# Autodesk Inventor assembly: IntakeExtensionBar
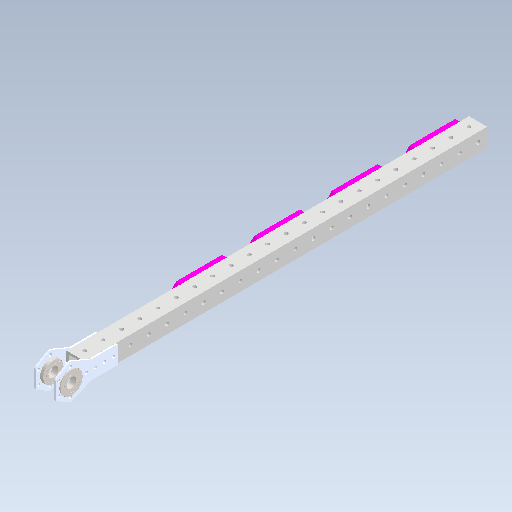
[picture p0: Inventor's stored thumbnail of the model, 512x512]
Saved by Autodesk Inventor 2020 (Build 240168000, 168)
## iProperties
Created: 2020-01-19
Part Number: IntakeExtensionBar
Document SubType Name: Assembly
Designer: srini
Author: srini
## Documents named in this file (5)
- C:\Users\srini\Documents\FRC\2020\IntakeShooter\IntakeExtensionBar.iam
- C:\Users\srini\Documents\FRC\2020\IntakeShooter\1x1x18.ipt
- C:\Users\srini\Documents\FRC\2020\IntakeShooter\VersaFrame_End_Bearing_Gusset_217-3554.ipt
- C:\Users\srini\Documents\FRC\2020\IntakeShooter\13_75mm_1_2_ThunderHex_ID_x_1_125_OD_x_0_313_WD_Flanged_Bearing_217-4006.ipt
- C:\Users\srini\Documents\FRC\2020\IntakeShooter\ShaftRest.ipt
## Components (9 placed, 4 different names)
1. 1x1x18:1 — Insert:7, Insert:8, Insert:9, Insert:10, Insert:11, Insert:12, Insert:13, Insert:14, Insert:15, Insert:16, Insert:17, Insert:18, Insert:19
2. VersaFrame_End_Bearing_Gusset_217-3554:1 — Insert:5, Insert:16, Insert:17
3. VersaFrame_End_Bearing_Gusset_217-3554:2 — Insert:6, Insert:18, Insert:19
4. 13_75mm_1_2_ThunderHex_ID_x_1_125_OD_x_0_313_WD_Flanged_Bearing_217-4006:1 — Insert:5
5. 13_75mm_1_2_ThunderHex_ID_x_1_125_OD_x_0_313_WD_Flanged_Bearing_217-4006:2 — Insert:6
6. ShaftRest:1 — Insert:7, Insert:8, Insert:11
7. ShaftRest:2 — Insert:9, Insert:12
8. ShaftRest:3 — Insert:10, Insert:13
9. ShaftRest:4 — Insert:14, Insert:15
## Relationships (15: Insert 15)
- Insert:5: VersaFrame_End_Bearing_Gusset_217-3554:1 ↔ 13_75mm_1_2_ThunderHex_ID_x_1_125_OD_x_0_313_WD_Flanged_Bearing_217-4006:1
- Insert:6: VersaFrame_End_Bearing_Gusset_217-3554:2 ↔ 13_75mm_1_2_ThunderHex_ID_x_1_125_OD_x_0_313_WD_Flanged_Bearing_217-4006:2
- Insert:7: 1x1x18:1 ↔ ShaftRest:1
- Insert:8: 1x1x18:1 ↔ ShaftRest:1
- Insert:9: 1x1x18:1 ↔ ShaftRest:2
- Insert:10: 1x1x18:1 ↔ ShaftRest:3
- Insert:11: 1x1x18:1 ↔ ShaftRest:1
- Insert:12: 1x1x18:1 ↔ ShaftRest:2
- Insert:13: 1x1x18:1 ↔ ShaftRest:3
- Insert:14: 1x1x18:1 ↔ ShaftRest:4
- Insert:15: 1x1x18:1 ↔ ShaftRest:4
- Insert:16: 1x1x18:1 ↔ VersaFrame_End_Bearing_Gusset_217-3554:1
- Insert:17: 1x1x18:1 ↔ VersaFrame_End_Bearing_Gusset_217-3554:1
- Insert:18: 1x1x18:1 ↔ VersaFrame_End_Bearing_Gusset_217-3554:2
- Insert:19: 1x1x18:1 ↔ VersaFrame_End_Bearing_Gusset_217-3554:2
